# Autodesk Inventor assembly: GEABP0.5-24-3-B-3
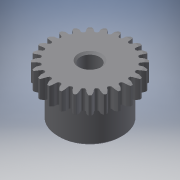
[picture p0: Inventor's stored thumbnail of the model, 180x180]
Saved by Autodesk Inventor 2019 (Build 230136000, 136)
## iProperties
Category: PARTsolutions
Company: MISUMI
Created: 2024-02-14
Part Number: GEABP0.5-24-3-B-3
Catalog Web Link: www.cadenas.de
Description: GEABM, GEABMS, GEABMT, GEABP, GEABPS, GEABPT, GEABA, GEABAS, GEABAT-Plastic Spur Gears - Pressure Angle 20 Degrees, Module 0.5/0.8/1.0/1.5/2.0/2.5/3.0
Vendor: MISUMI
Document SubType Name: Assembly
Designer: psAdmin
Manufacturer: MISUMI
Mass: 0.665819 g
Surface Area: 7.08795 cm^2
Volume: 0.665819 cm^3
Density: 1 g/cm^3
Title: GEABP0.5-24-3-B-3
Author: Cadenas PARTsolutions
Comments: Plastic Spur Gears - Pressure Angle 20 Degrees, Module 0.5/0.8/1.0/1.5/2.0/2.5/3.0
PSOL_IDENT_0: {$CADENAS_DATA/23d-libs/misumi/metric/54_spur_gears/geabms20_asmtab.prj},393 {VTYP=3D},{STYP=ASSTAB}
PSOL_IDENT_1: ,{NB=GEABP0.5-24-3-B-3},{LINA=GEABP0.5-24-3-B-3},{NN=GEABM, GEABMS, GEABMT, GEABP, GEABPS, GEABPT, G
PSOL_IDENT_2: EABA, GEABAS, GEABAT},{DATE=13.11.2023 01:04:12},{GEOMDATE=12.11.2023 05:54:43},{VERSION=},{LINEID=1
PSOL_IDENT_3: 0},{WBVAR=MATSG,MATCR,NT,B,TS,PS,ALT1,ALT2,TPC,ALT11,ALT10,BS,ALT3,Z,J,ALT4,Q,R,S,T,ALT5,LFC,LTC,MAL
PSOL_IDENT_4: T5,ALT6,KFC,KTC,K},{WBNUMERIC=NT,B,BS,Z,J,Q,R,S,T,LFC,LTC,KFC,KTC,K}  {NB=GEABP0.5-24-3-B-3},{LINA=G
PSOL_IDENT_5: EABP0.5-24-3-B-3},{KT=DUMMY},{PN=GEABP0.5-24-3-B-3},{TYPE=GEABP},{MATSG=PW},{MATSGALG='MCN','MC Nylo
PSOL_IDENT_6: n','PW','Polyacetal White','PB','Polyacetal Blue'},{MATCR=},{MATCRALG='','-'},{MOD=0.5},{MOD1=0.5},{
PSOL_IDENT_7: NT=24},{NTALG=15,16,18,20,24,25,28,30,32,36,40,45,48,50,56,60,64,70,72,80,90,100,120},{B=3},{BALG=3,
PSOL_IDENT_8: 5},{TS=B},{TSALG='B','B'},{TSPN=-B},{PS=3},{PSALG='3','3','4','4','5','5','6','6','7','7'},{PSCRL='3'
PSOL_IDENT_9: ,'3','4','4','5','5','6','6','7','7'},{PSCRW='0','0'},{DD=12.0},{DD05=12},{DD08=19.2},{DD10=24},{DD1
PSOL_IDENT_10: 5=36},{DD20=48},{DD25=60},{DD30=72},{D=13.0},{D05=13},{D08=20.8},{D10=26},{D15=39},{D20=52},{D25=65}
PSOL_IDENT_11: ,{D30=78},{G=10.75},{G05=10.75},{G08=17.2},{G10=21.5},{G15=32.25},{G20=43},{G25=53.75},{G30=64.5},{H=
PSOL_IDENT_12: 10.0},{L=8},{LL1=5},{LL2=2.5},{M=M3},{M3D=3},{P=3.00},{DD1=0},{CIFR=8.8},{CIFM=3},{CIFK=0},{CIFTAP=1
PSOL_IDENT_13: },{SCREW=3.000},{SCREWL=3.000},{ALT1=},{ALT1ALG='','w/o Set Screw','KC90','with KC90 (Set Screw)','K
PSOL_IDENT_14: C120','with KC120 (Set Screw)'},{ALT1PN=},{ALT2=},{ALT2ALG='','w/o TPC (Tapped Hole Dimension)','TPC'
PSOL_IDENT_15: ,'with TPC (Tapped Hole Dimension)'},{TPC=N/A},{TPCALG='N/A'},{ALT2PN=},{KC=0},{ALT11=},{ALT11ALG=''
PSOL_IDENT_16: ,'Not applicable'},{ALT11PN=},{DEG=0},{ALT10=},{ALT10ALG= '','w/o BS (Boss Cut)','BS','with BS (Boss
PSOL_IDENT_17: Cut)' },{ALT10PN=},{BS=0.0},{BSALG=0},{BSMIN=6.000},{BSMINALG=6},{BSMAX=5},{LL13D=5},{LL23D=5.5},{A
PSOL_IDENT_18: LT3=},{ALT3ALG= '','w/o Stepped Hole','DHR','with DHR (Stepped Hole)' },{ALT3PN=},{ZJPN=},{ALT31=0},
PSOL_IDENT_19: {ALT32=1},{Z=0},{ZALG=0},{ZMINL=5},{ZMAXL=6},{ZMINR=5},{ZMAXR=6},{ZPN=},{J=0.0},{JALG=0},{JMIN=2},{J
PSOL_IDENT_20: MAX=0},{JPN=},{ALT4=},{ALT4ALG= '','Not applicable' },{ALT4PN=},{QRSTPN=},{LB=8.000},{Q=0},{QALG=0},
PSOL_IDENT_21: {QMIN=5},{QMAX=6},{QPN=},{R=0},{RALG=0},{RMIN=5},{RMAX=6},{RPN=},{S=0},{SALG=0},{SMIN=3},{SMAX=2},{S
PSOL_IDENT_22: PN=},{T=0},{TALG=0},{TMIN=3},{TMAX=0},{TPN=},{ALT5=},{ALT5ALG= '','Not applicable' },{LFC=0},{LFCALG=
PSOL_IDENT_23: 0},{LTC=0},{LTCALG=0},{LPCDMIN=11},{LPCDMAX=3},{LCMAX=6},{MALT5=N/A},{MALT5ALG= 'N/A' },{LCMAX2=3},{
PSOL_IDENT_24: C=0.0},{ALT5PN=},{ALT6=},{ALT6ALG= '','Not applicable' },{ALT6PN=},{KFTCPN=},{KFC=0},{KFCALG=[0]},{K
PSOL_IDENT_25: FCPN=},{KTC=0},{KTCALG=[0]},{KTCPN=},{KPCDMIN1=10},{KPCDMAX1=3},{KPCDMIN2=17},{KPCDMAX2=3},{K=0.0},{
PSOL_IDENT_26: KALG=[0]},{KPCD=0},{KPN=},{AG=0},{LBS=8},{PCD=0},{SHN=0},{SHDEG1=0},{SHDEG2=0},{PZQRDD2=3},{PPATH=ge
PSOL_IDENT_27: abms20/geabms20_asmtpl.prj}
NB: GEABP0.5-24-3-B-3
NN: GEABM, GEABMS, GEABMT, GEABP, GEABPS, GEABPT, GEABA, GEABAS, GEABAT
NT: 24
NBSYN: $PN.
LINA: GEABP0.5-24-3-B-3
CATALOG: Misumi
PN: GEABP0.5-24-3-B-3
MATSG: Polyacetal White
MATCR: -
MOD: 0.5
B: 3
TS: B
PS: 3
DD: 12
D: 13
G: 10.75
H: 10
L: 8
LL1: 5
LL2: 2.5
M: M3
DD1: 0
ALT1: w/o Set Screw
ALT2: w/o TPC (Tapped Hole Dimension)
TPC: N/A
ALT11: Not applicable
ALT10: w/o BS (Boss Cut)
BS: 0
ALT3: w/o Stepped Hole
Z: 0
J: 0
ALT4: Not applicable
Q: 0
R: 0
S: 0
T: 0
ALT5: Not applicable
LFC: 0
LTC: 0
MALT5: N/A
C: 0
ALT6: Not applicable
KFC: 0
KTC: 0
K: 0
SUPPLIER: MISUMI
ARTICLENO: GEABP0.5-24-3-B-3
BOMINFO: GEABP0.5-24-3-B-3
CREATOR: CADENAS GmbH
## Documents named in this file (3)
- e:\temp\worker_COMMON_2\temp\tmp_6768_84_sWLUN\format_0\GEABP0_5-24-3-B-3.iam
- e:\temp\worker_COMMON_2\temp\tmp_6768_84_sWLUN\format_0\GEABP0_5-24-3-B-3_b.ipt
- e:\temp\worker_COMMON_2\temp\tmp_6768_84_sWLUN\format_0\SET-SCREW3-3.ipt
## Components (2 placed, 2 different names)
1. GEABP0_5-24-3-B-3_b:1 — gear_to_screw_XY@1 <-> CP_XY@2, gear_to_screw_Z@1 <-> CP_Z@2, gear_to_screw_YZ@1 <-> CP_YZ@2
2. SET-SCREW3-3:1 — gear_to_screw_XY@1 <-> CP_XY@2, gear_to_screw_Z@1 <-> CP_Z@2, gear_to_screw_YZ@1 <-> CP_YZ@2
## Relationships (3: Mate 2, Angle 1)
- gear_to_screw_XY@1 <-> CP_XY@2 [Mate]: GEABP0_5-24-3-B-3_b:1 ↔ SET-SCREW3-3:1
- gear_to_screw_Z@1 <-> CP_Z@2 [Mate]: GEABP0_5-24-3-B-3_b:1 ↔ SET-SCREW3-3:1
- gear_to_screw_YZ@1 <-> CP_YZ@2 [Angle] (0 deg): GEABP0_5-24-3-B-3_b:1 ↔ SET-SCREW3-3:1
